# Autodesk Inventor assembly: simpleste Anbindung
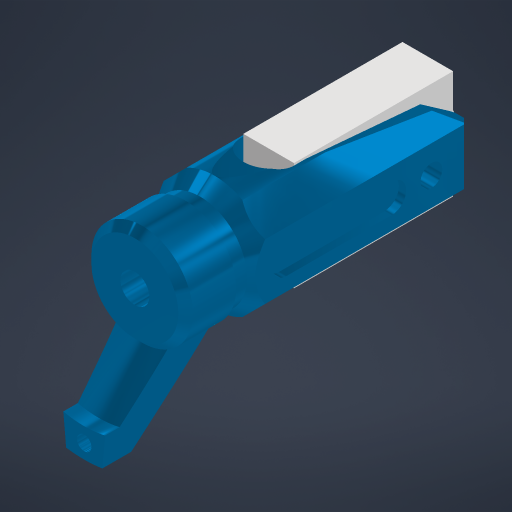
[picture p0: Inventor's stored thumbnail of the model, 512x512]
Saved by Autodesk Inventor 2023.2 (Build 272271000, 271)
## iProperties
Created: 2023-04-05
Part Number: simpleste Anbindung
Document SubType Name: Assembly
Designer: tadeus
Author: tadeus
## Documents named in this file (3)
- C:\Users\tadeu\Documents\0 Nerdy\CAD\Inventor\Studium\5. Semester\NWPL\WKA\simpleste Anbindung.iam
- C:\Users\tadeu\Documents\0 Nerdy\CAD\Inventor\Studium\5. Semester\NWPL\WKA\simpleste Anbindung.ipt
- C:\Users\tadeu\Documents\0 Nerdy\CAD\Inventor\Studium\5. Semester\NWPL\WKA\RotorArm.ipt
## Components (2 placed, 2 different names)
1. simpleste Anbindung:1 — Fluchtend:1, Passend:1, Tangential:1
2. RotorArm:1 — Fluchtend:1, Passend:1, Tangential:1
## Relationships (3: Flush 1, Mate 1, Tangent 1)
- Fluchtend:1 [Flush]: simpleste Anbindung:1 ↔ RotorArm:1
- Passend:1 [Mate]: simpleste Anbindung:1 ↔ RotorArm:1
- Tangential:1: simpleste Anbindung:1 ↔ RotorArm:1
